# Autodesk Inventor assembly: NONE
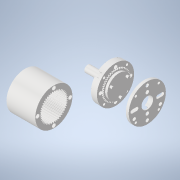
[picture p0: Inventor's stored thumbnail of the model, 180x180]
Saved by Autodesk Inventor 2022.3 (Build 263350000, 350)
## iProperties
Created: 2022-06-19
Part Number: NONE
Document SubType Name: Assembly
Designer: YusukeKunita
Author: YusukeKunita
Revision Number: NONE
## Documents named in this file (5)
- C:\Users\YusukeKunita\Desktop\IG32-step\IG32_step\IG32_100\NONE.iam
- C:\Users\YusukeKunita\Desktop\IG32-step\IG32_step\IG32_100\Part 1_4.ipt
- C:\Users\YusukeKunita\Desktop\IG32-step\IG32_step\IG32_100\Part 1_5.ipt
- C:\Users\YusukeKunita\Desktop\IG32-step\IG32_step\IG32_100\Part 1_6.ipt
- C:\Users\YusukeKunita\Desktop\IG32-step\IG32_step\IG32_100\Part 1_7.ipt
## Components (4 placed, 4 different names)
1. NAUO1
2. NAUO2 — 回転:1
3. NAUO3
4. Part 1_7:1 — 回転:1
## Relationships (1: RevoluteJoint 1)
- 回転:1 [RevoluteJoint]: NAUO2 ↔ Part 1_7:1
